# Autodesk Inventor assembly: CORE
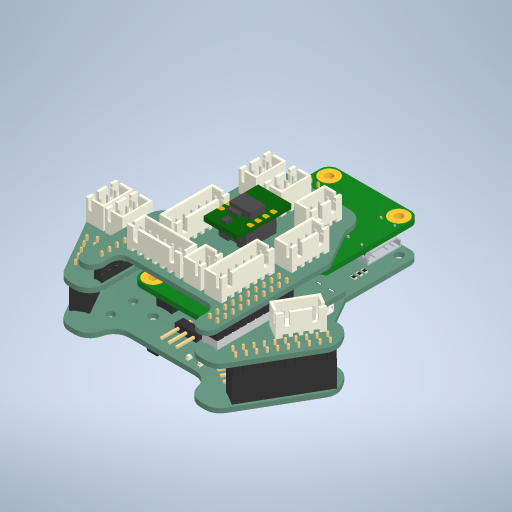
[picture p0: Inventor's stored thumbnail of the model, 512x512]
Saved by Autodesk Inventor 2024.1 (Build 281209000, 209)
## iProperties
Created: 2025-04-22
Part Number: CORE
Document SubType Name: Assembly
Designer: hibik
Author: hibik
## Documents named in this file (5)
- C:\Users\hibik\Documents\Robomech\RESCUE\ORCA\hard\board\CORE_model\CORE.iam
- C:\Users\hibik\Documents\Robomech\RESCUE\ORCA\hard\board\CORE_model\cpu.iam
- C:\Users\hibik\Documents\Robomech\RESCUE\ORCA\hard\board\CORE_model\cpu_hat_left.iam
- C:\Users\hibik\Documents\Robomech\RESCUE\ORCA\hard\board\CORE_model\cpu_hat_right.iam
- C:\Users\hibik\Documents\Robomech\RESCUE\ORCA\hard\board\CORE_model\cpu_hat_upper.iam
## Components (4 placed, 4 different names)
1. cpu:1 [sub-assembly] — フラッシュ:1, フラッシュ:2, メイト:1, フラッシュ:3, フラッシュ:4, メイト:2, フラッシュ:5, フラッシュ:6
2. cpu_hat_left:1 [sub-assembly] — メイト:2, フラッシュ:5, フラッシュ:6
3. cpu_hat_right:1 [sub-assembly] — メイト:1, フラッシュ:3, フラッシュ:4, メイト:3, フラッシュ:7, フラッシュ:8
4. cpu_hat_upper:1 [sub-assembly] — メイト:3, フラッシュ:7, フラッシュ:8
## Relationships (11: Flush 8, Mate 3)
- フラッシュ:1 [Flush]: cpu:1
- フラッシュ:2 [Flush]: cpu:1
- メイト:1 [Mate]: cpu:1 ↔ cpu_hat_right:1
- フラッシュ:3 [Flush]: cpu:1 ↔ cpu_hat_right:1
- フラッシュ:4 [Flush]: cpu:1 ↔ cpu_hat_right:1
- メイト:2 [Mate]: cpu:1 ↔ cpu_hat_left:1
- フラッシュ:5 [Flush]: cpu:1 ↔ cpu_hat_left:1
- フラッシュ:6 [Flush]: cpu:1 ↔ cpu_hat_left:1
- メイト:3 [Mate]: cpu_hat_right:1 ↔ cpu_hat_upper:1
- フラッシュ:7 [Flush]: cpu_hat_right:1 ↔ cpu_hat_upper:1
- フラッシュ:8 [Flush]: cpu_hat_right:1 ↔ cpu_hat_upper:1
